# Autodesk Inventor assembly: C-AFBD11-15
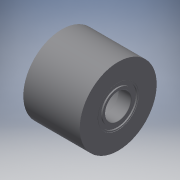
[picture p0: Inventor's stored thumbnail of the model, 180x180]
Saved by Autodesk Inventor 2019 (Build 230136000, 136)
## iProperties
Category: PARTsolutions
Company: MISUMI
Created: 2023-11-09
Part Number: C-AFBD11-15
Catalog Web Link: www.cadenas.de
Description: C-AFBD, C-AFDF-Economy Idlers Backside Tension Type
Vendor: MISUMI
Document SubType Name: Assembly
Designer: psAdmin
Manufacturer: MISUMI
Mass: 1.60086 g
Surface Area: 14.1557 cm^2
Volume: 1.60086 cm^3
Density: 1 g/cm^3
Title: C-AFBD11-15
Author: Cadenas PARTsolutions
Comments: Economy Idlers Backside Tension Type
PSOL_IDENT_0: {$CADENAS_DATA/23d-libs/misumi/metric/51_timing_pulleys/c_afbd_asmtab.prj},191 {VTYP=3D},{STYP=ASSTA
PSOL_IDENT_1: B},{NB=C-AFBD11-15},{LINA=C-AFBD11-15},{NN=C-AFBD, C-AFDF},{DATE=13.09.2022 06:49:12},{GEOMDATE=18.0
PSOL_IDENT_2: 5.2021 06:13:57},{VERSION=},{LINEID=30},{WBVAR=TS,TYPE},{WBNUMERIC=}  {NB=C-AFBD11-15},{LINA=C-AFBD1
PSOL_IDENT_3: 1-15},{KT=DUMMY},{PN=C-AFBD11-15},{TS=BSB},{TSALG= 'CB','Center Bearing Type','BSB','Both Sides Bear
PSOL_IDENT_4: ing Type' },{TYPE=C-AFBD},{TYPEALG= 'C-AFBD','No Flange','C-AFDF','Flanged' },{W=11.0},{NOM=15},{D=1
PSOL_IDENT_5: 5},{F=18},{A=7.0},{ABI=-},{ABM=60},{S=0.00},{NO=675ZZx2},{BN=696},{DD=5},{B=2.5},{RR=-},{E=20.000},{
PSOL_IDENT_6: BD=15},{DH=13.400},{DD2=15.7},{RTT=1.000},{PTT=1.000},{CIF=0.000},{PPATH=c_afbd/c_afbd_asmtpl.prj}
NB: C-AFBD11-15
NN: C-AFBD, C-AFDF
NT: Economy Idlers Backside Tension Type
NBSYN: $PN.
LINA: C-AFBD11-15
CATALOG: Misumi
PN: C-AFBD11-15
TS: Both Sides Bearing Type
TYPE: No Flange
W: 11
NOM: 15
D: 15
F: 18
A: 7
ABI: -
ABM: 60
S: 0
NO: 675ZZx2
DD: 5
B: 2.5
RR: -
SUPPLIER: MISUMI
ARTICLENO: C-AFBD11-15
BOMINFO: C-AFBD11-15
CREATOR: CADENAS GmbH
## Documents named in this file (3)
- e:\temp\worker_COMMON_2\temp\tmp_4572_108_6i364\format_0\C-AFBD11-15.iam
- e:\temp\worker_COMMON_2\temp\tmp_4572_108_6i364\format_0\C-AFBD11-15_bw.ipt
- e:\temp\worker_COMMON_2\temp\tmp_4572_108_6i364\format_0\bearing_675.ipt
## Components (3 placed, 2 different names)
1. C-AFBD11-15_bw:1 — b600_1_XY@1 <-> to_housing_center_XY@2, b600_1_Z@1 <-> to_housing_center_Z@2, b600_1_YZ@1 <-> to_housing_center_YZ@2, b600_2_XY@1 <-> to_housing_center_XY@3, b600_2_Z@1 <-> to_housing_center_Z@3, b600_2_YZ@1 <-> to_housing_center_YZ@3
2. bearing_675:1 — b600_1_XY@1 <-> to_housing_center_XY@2, b600_1_Z@1 <-> to_housing_center_Z@2, b600_1_YZ@1 <-> to_housing_center_YZ@2
3. bearing_675:2 — b600_2_XY@1 <-> to_housing_center_XY@3, b600_2_Z@1 <-> to_housing_center_Z@3, b600_2_YZ@1 <-> to_housing_center_YZ@3
## Relationships (6: Mate 4, Angle 2)
- b600_1_XY@1 <-> to_housing_center_XY@2 [Mate]: C-AFBD11-15_bw:1 ↔ bearing_675:1
- b600_1_Z@1 <-> to_housing_center_Z@2 [Mate]: C-AFBD11-15_bw:1 ↔ bearing_675:1
- b600_1_YZ@1 <-> to_housing_center_YZ@2 [Angle] (0 deg): C-AFBD11-15_bw:1 ↔ bearing_675:1
- b600_2_XY@1 <-> to_housing_center_XY@3 [Mate]: C-AFBD11-15_bw:1 ↔ bearing_675:2
- b600_2_Z@1 <-> to_housing_center_Z@3 [Mate]: C-AFBD11-15_bw:1 ↔ bearing_675:2
- b600_2_YZ@1 <-> to_housing_center_YZ@3 [Angle] (0 deg): C-AFBD11-15_bw:1 ↔ bearing_675:2
